# Autodesk Inventor assembly: chain
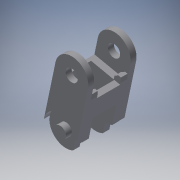
[picture p0: Inventor's stored thumbnail of the model, 180x180]
Saved by Autodesk Inventor 2019.3 (Build 233278000, 278)
## iProperties
Created: 2020-08-28
Part Number: chain
Material: Generisch
Document SubType Name: Assembly
Designer: Nicolas Frick
Author: Nicolas Frick
## Documents named in this file (3)
- C:\Users\Nicolas Frick\Sync\OneDrive\airhockeybot\mechanical_design\inventor\Chain\chain.iam
- C:\Users\Nicolas Frick\Sync\OneDrive\airhockeybot\mechanical_design\inventor\Chain\chain_elmt_1.ipt
- C:\Users\Nicolas Frick\Sync\OneDrive\airhockeybot\mechanical_design\inventor\Chain\chain_elmt_2.ipt
## Components (3 placed, 2 different names)
1. chain_elmt_1:1 — Passend:3, Passend:4, Fluchtend:2
2. chain_elmt_1:2 — Passend:1, Fluchtend:1, Passend:2, Passend:3
3. chain_elmt_2:1 — Passend:1, Fluchtend:1, Passend:2, Passend:4, Fluchtend:2
## Relationships (6: Mate 4, Flush 2)
- Passend:1 [Mate]: chain_elmt_1:2 ↔ chain_elmt_2:1
- Fluchtend:1 [Flush]: chain_elmt_1:2 ↔ chain_elmt_2:1
- Passend:2 [Mate] (5 mm): chain_elmt_1:2 ↔ chain_elmt_2:1
- Passend:3 [Mate]: chain_elmt_1:1 ↔ chain_elmt_1:2
- Passend:4 [Mate]: chain_elmt_1:1 ↔ chain_elmt_2:1
- Fluchtend:2 [Flush]: chain_elmt_1:1 ↔ chain_elmt_2:1
